# Autodesk Inventor assembly: plateCam
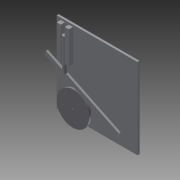
[picture p0: Inventor's stored thumbnail of the model, 180x180]
Saved by Autodesk Inventor 2015 (Build 190159000, 159)
## iProperties
Created: 2015-04-14
Part Number: plateCam
Document SubType Name: Assembly
Designer: WASHHSST
Author: WASHHSST
## Documents named in this file (5)
- C:\Users\washhsst\Documents\GitHub\myWork\plateCam\plateCam.iam
- C:\Users\washhsst\Documents\GitHub\myWork\plateCam\Base.ipt
- C:\Users\washhsst\Documents\GitHub\myWork\plateCam\plateCam\Design Accelerator\Disc Cam4.iam
- C:\Users\washhsst\Documents\GitHub\myWork\plateCam\Part7.ipt
- C:\Users\washhsst\Documents\GitHub\myWork\plateCam\Part8.ipt
## Components (4 placed, 4 different names)
1. Base:1 — Mate:1, Mate:2, Mate:3, Mate:4, Tangent:2, Tangent:3
2. Disc Cam:1 [sub-assembly] — Mate:1, Mate:2, Tangent:1
3. Part7:1 — Mate:3, Tangent:1, Mate:4, Mate:5
4. Part8:1 — Tangent:2, Tangent:3, Mate:5
## Relationships (8: Mate 5, Tangent 3)
- Mate:1: Base:1 ↔ Disc Cam:1
- Mate:2: Base:1 ↔ Disc Cam:1
- Mate:3: Base:1 ↔ Part7:1
- Tangent:1: Disc Cam:1 ↔ Part7:1
- Mate:4: Base:1 ↔ Part7:1
- Tangent:2: Base:1 ↔ Part8:1
- Tangent:3: Base:1 ↔ Part8:1
- Mate:5: Part7:1 ↔ Part8:1
